# Autodesk Inventor assembly: ensamble_final
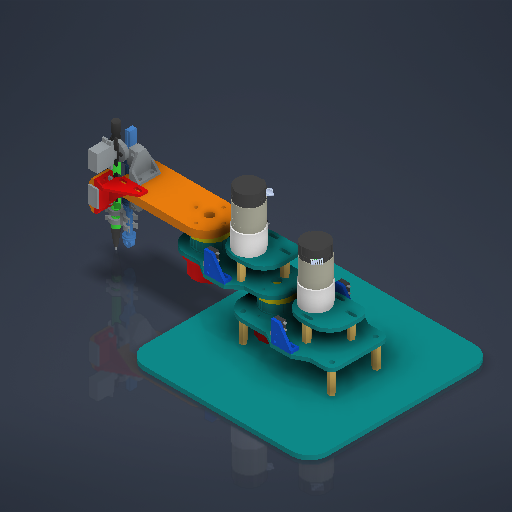
[picture p0: Inventor's stored thumbnail of the model, 512x512]
Saved by Autodesk Inventor 2026.2 (Build 302298000, 298)
## iProperties
Created: 2024-10-02
Part Number: ensamble_final
Document SubType Name: Assembly
Designer: User
Author: User
## Documents named in this file (6)
- C:\Users\User\OneDrive - Universidad EIA\Documentos\Universidad Octavo Semestre\Robotica Industrial\matlab\SCARA\mariana_scara_final\mariana_scara_final\ensamble_final.iam
- C:\Users\User\OneDrive - Universidad EIA\Documentos\Universidad Octavo Semestre\Robotica Industrial\matlab\SCARA\mariana_scara_final\mariana_scara_final\base_final.iam
- C:\Users\User\OneDrive - Universidad EIA\Documentos\Universidad Octavo Semestre\Robotica Industrial\matlab\SCARA\mariana_scara_final\mariana_scara_final\eje.iam
- C:\Users\User\OneDrive - Universidad EIA\Documentos\Universidad Octavo Semestre\Robotica Industrial\matlab\SCARA\mariana_scara_final\mariana_scara_final\BaseSuperior_final.iam
- C:\Users\User\OneDrive - Universidad EIA\Documentos\Universidad Octavo Semestre\Robotica Industrial\matlab\SCARA\mariana_scara_final\mariana_scara_final\herramienta_final.iam
- C:\Users\User\OneDrive - Universidad EIA\Documentos\Universidad Octavo Semestre\Robotica Industrial\matlab\SCARA\mariana_scara_final\mariana_scara_final\lapiz.ipt
## Components (6 placed, 5 different names)
1. base_final:1 [sub-assembly] — Mate:1, Flush:1, Flush:4
2. eje:1 [sub-assembly] — Mate:1, Flush:1, Mate:2, Mate:3, Mate:4, Mate:5, Mate:6
3. BaseSuperior_final:1 [sub-assembly] — Mate:2, Mate:3, Mate:4, Mate:5, Mate:6, Flush:2, Mate:7
4. eje:2 [sub-assembly] — Flush:2, Mate:7, Mate:8, Mate:9, Mate:10, Mate:11, Mate:12
5. herramienta_final:1 [sub-assembly] — Mate:8, Mate:9, Mate:10, Mate:11, Mate:12, Mate:13, Mate:14
6. lapiz:1 — Flush:3, Mate:13
## Relationships (18: Mate 14, Flush 4)
- Mate:1: base_final:1 ↔ eje:1
- Flush:1 (-23.507 mm): base_final:1 ↔ eje:1
- Mate:2: eje:1 ↔ BaseSuperior_final:1
- Mate:3: eje:1 ↔ BaseSuperior_final:1
- Mate:4: eje:1 ↔ BaseSuperior_final:1
- Mate:5: eje:1 ↔ BaseSuperior_final:1
- Mate:6: eje:1 ↔ BaseSuperior_final:1
- Flush:2 (-23.507 mm): BaseSuperior_final:1 ↔ eje:2
- Mate:7: BaseSuperior_final:1 ↔ eje:2
- Mate:8: eje:2 ↔ herramienta_final:1
- Mate:9: eje:2 ↔ herramienta_final:1
- Mate:10: eje:2 ↔ herramienta_final:1
- Mate:11: eje:2 ↔ herramienta_final:1
- Mate:12: eje:2 ↔ herramienta_final:1
- Flush:3 (-47.3 mm): lapiz:1
- Mate:13: herramienta_final:1 ↔ lapiz:1
- Mate:14 (25 mm): herramienta_final:1
- Flush:4 (-125 mm): base_final:1
